# Autodesk Inventor assembly: Cabos
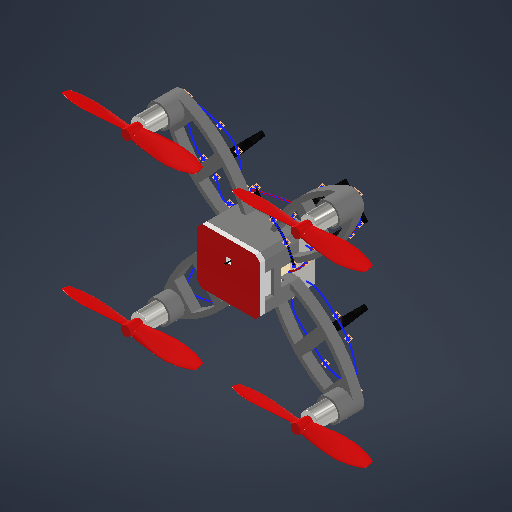
[picture p0: Inventor's stored thumbnail of the model, 512x512]
Saved by Autodesk Inventor 2027 (Build 310192000, 192)
## iProperties
Created: 2026-07-18
Part Number: Cabos
Document SubType Name: Assembly
Designer: marcu
Mass: 19.2027 g
Surface Area: 228.132 cm^2
Volume: 19.2027 cm^3
Density: 1 g/cm^3
Author: marcu
## Documents named in this file (3)
- C:\Users\marcu\projetos\cin-maker\Projeto_drone\Cabos.iam
- C:\Users\marcu\projetos\cin-maker\Projeto_drone\Montagem_Drone1.iam
- C:\Users\marcu\projetos\cin-maker\Projeto_drone\Cabos\AIP\Cabeamento elétrico\Cabos.Fiação6.iam
## Components (2 placed, 2 different names)
1. Montagem_Drone1:1 [sub-assembly]
2. Fiação6 [sub-assembly]
## Named parameters: Finish1_Area = 0.843806, Finish1_Thickness = 0.008 mm, Finish2_Area = 0.807012, Finish2_Thickness = 0.008 mm, Finish3_Area = 0.7799, Finish3_Thickness = 0.008 mm, Finish4_Area = 0.814304, Finish4_Thickness = 0.008 mm, Finish5_Area = 1.11135, Finish5_Thickness = 0.008 mm, Finish6_Area = 1.04303, Finish6_Thickness = 0.008 mm
note: some values were not read from the file. Shown as the stored number, unit unknown: "Finish1_Area", "Finish2_Area", "Finish3_Area", "Finish4_Area", "Finish5_Area", "Finish6_Area".
